# Autodesk Inventor assembly: Servo
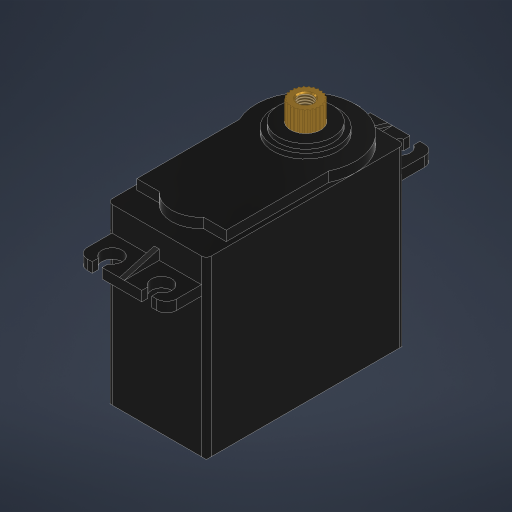
[picture p0: Inventor's stored thumbnail of the model, 512x512]
Saved by Autodesk Inventor 2023.2 (Build 272271000, 271)
## iProperties
Created: 2023-04-06
Part Number: Servo
Document SubType Name: Assembly
Designer: tadeus
Author: tadeus
## Documents named in this file (3)
- C:\Users\tadeu\Documents\0 Nerdy\CAD\Inventor\Studium\5. Semester\NWPL\WKA\Bauteile\Technik\Servo\Servo.iam
- C:\Users\tadeu\Documents\0 Nerdy\CAD\Inventor\Studium\5. Semester\NWPL\WKA\Bauteile\Technik\Servo\Servo.ipt
- C:\Users\tadeu\Documents\0 Nerdy\CAD\Inventor\Studium\5. Semester\NWPL\WKA\Bauteile\Technik\Servo\Zahnrad Servo.ipt
## Components (2 placed, 2 different names)
1. Servo:1 — Drehbar:1
2. Zahnrad Servo:1 — Drehbar:1
## Relationships (1: RevoluteJoint 1)
- Drehbar:1 [RevoluteJoint] (3 mm): Servo:1 ↔ Zahnrad Servo:1
